# Autodesk Inventor assembly: v1.0
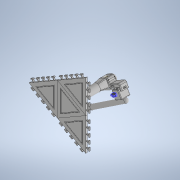
[picture p0: Inventor's stored thumbnail of the model, 180x180]
Saved by Autodesk Inventor 2022.3 (Build 263350000, 350)
## iProperties
Created: 2023-03-28
Part Number: v1.0
Document SubType Name: Assembly
Designer: Manuel Hueso Béjar
Author: Manuel Hueso Béjar
## Documents named in this file (13)
- C:\Users\Manuel Hueso Béjar\Desktop\3\2º Cuatrimestre\Robótica\Trabajo\v1.0\v1.0.iam
- C:\Users\Manuel Hueso Béjar\Desktop\3\2º Cuatrimestre\Robótica\Trabajo\v1.0\Base.ipt
- C:\Users\Manuel Hueso Béjar\Downloads\nema-17-motor-a-pasos-17hs4401-1-7amp-4kg-cm-1.snapshot.4\Nema 17 Motor a Pasos 17HS4401.iam
- C:\Users\Manuel Hueso Béjar\Desktop\3\2º Cuatrimestre\Robótica\Trabajo\v1.0\Base2.ipt
- C:\Users\Manuel Hueso Béjar\Desktop\3\2º Cuatrimestre\Robótica\Trabajo\v1.0\Tube_1.ipt
- C:\Users\Manuel Hueso Béjar\Desktop\3\2º Cuatrimestre\Robótica\Trabajo\v1.0\Tube_2.ipt
- C:\Users\Manuel Hueso Béjar\Desktop\3\2º Cuatrimestre\Robótica\Trabajo\v1.0\Joint_Tubes_1_2.ipt
- C:\Users\Manuel Hueso Béjar\Downloads\timing-pulley-gt2-16-teeth-5mm-bore-2.snapshot.7\GT2-16T\GT2_16T.ipt
- C:\Users\Manuel Hueso Béjar\Desktop\3\2º Cuatrimestre\Robótica\Trabajo\v1.0\Rod_1.ipt
- C:\Users\Manuel Hueso Béjar\Downloads\rolling-bearing-lmxxuu-1.snapshot.6\roulement lmxxuu (ap203).ipt
- C:\Users\Manuel Hueso Béjar\Desktop\3\2º Cuatrimestre\Robótica\Trabajo\v1.0\Joint_Bearings.ipt
- C:\Users\Manuel Hueso Béjar\Downloads\sg90-micro-servo-9g-tower-pro-1.snapshot.3\SG90 - Micro Servo 9g - Tower Pro.1.ipt
- C:\Users\Manuel Hueso Béjar\Desktop\3\2º Cuatrimestre\Robótica\Trabajo\v1.0\Tube_3.ipt
## Components (19 placed, 12 different names)
1. Base:1 — Rigid:1, Rigid:2, Rigid:3, Rigid:4, Rotational:7
2. Nema 17 Motor a Pasos 17HS4401:1 [sub-assembly] — Rigid:1
3. Base2:1 — Rigid:2
4. Base2:2 — Rigid:3
5. Base2:3 — Rigid:4
6. Tube_1:1 — Mate:3, Rigid:5, Mate:4, Mate:5, Mate:6, Mate:7, Rotational:7
7. Nema 17 Motor a Pasos 17HS4401:2 [sub-assembly] — Mate:8, Mate:9, Mate:10, Rotational:6
8. Nema 17 Motor a Pasos 17HS4401:3 [sub-assembly] — Mate:3, Rigid:5, Rotational:2
9. Tube_2:1 — Rotational:6, Rigid:8
10. Joint_Tubes_1_2:1 — Mate:4, Rotational:3, Rotational:4
11. GT2_16T:1 — Rotational:2
12. Joint_Tubes_1_2:2 — Mate:5, Mate:6, Mate:7, Rotational:5
13. Rod_1:1 — Rotational:4, Cylindrical:2
14. Rod_1:2 — Rotational:3, Rotational:5, Cylindrical:1
15. roulement lmxxuu (ap203):1 — Cylindrical:1, Rigid:7
16. roulement lmxxuu (ap203):2 — Cylindrical:2, Rigid:6
17. Joint_Bearings:1 — Rigid:6, Rigid:7, Mate:8, Mate:9, Mate:10
18. SG90 - Micro Servo 9g - Tower Pro.1:1
19. Tube_3:1 — Rigid:8
## Relationships (24: WeldJoint 8, Mate 8, RevoluteJoint 6, CylindricalJoint 2)
- Rigid:1 [WeldJoint]: Base:1 ↔ Nema 17 Motor a Pasos 17HS4401:1
- Rigid:2 [WeldJoint]: Base:1 ↔ Base2:1
- Rigid:3 [WeldJoint]: Base:1 ↔ Base2:2
- Rigid:4 [WeldJoint]: Base:1 ↔ Base2:3
- Mate:3: Tube_1:1 ↔ Nema 17 Motor a Pasos 17HS4401:3
- Rigid:5 [WeldJoint]: Tube_1:1 ↔ Nema 17 Motor a Pasos 17HS4401:3
- Rotational:2 [RevoluteJoint] (2.65 mm): Nema 17 Motor a Pasos 17HS4401:3 ↔ GT2_16T:1
- Mate:4: Tube_1:1 ↔ Joint_Tubes_1_2:1
- Mate:5: Tube_1:1 ↔ Joint_Tubes_1_2:2
- Mate:6: Tube_1:1 ↔ Joint_Tubes_1_2:2
- Mate:7: Tube_1:1 ↔ Joint_Tubes_1_2:2
- Rotational:3 [RevoluteJoint]: Joint_Tubes_1_2:1 ↔ Rod_1:2
- Rotational:4 [RevoluteJoint]: Joint_Tubes_1_2:1 ↔ Rod_1:1
- Rotational:5 [RevoluteJoint]: Joint_Tubes_1_2:2 ↔ Rod_1:2
- Cylindrical:1: Rod_1:2 ↔ roulement lmxxuu (ap203):1
- Cylindrical:2: Rod_1:1 ↔ roulement lmxxuu (ap203):2
- Rigid:6 [WeldJoint]: roulement lmxxuu (ap203):2 ↔ Joint_Bearings:1
- Rigid:7 [WeldJoint]: roulement lmxxuu (ap203):1 ↔ Joint_Bearings:1
- Mate:8: Nema 17 Motor a Pasos 17HS4401:2 ↔ Joint_Bearings:1
- Mate:9: Nema 17 Motor a Pasos 17HS4401:2 ↔ Joint_Bearings:1
- Mate:10: Nema 17 Motor a Pasos 17HS4401:2 ↔ Joint_Bearings:1
- Rotational:6 [RevoluteJoint]: Nema 17 Motor a Pasos 17HS4401:2 ↔ Tube_2:1
- Rigid:8 [WeldJoint]: Tube_2:1 ↔ Tube_3:1
- Rotational:7 [RevoluteJoint]: Base:1 ↔ Tube_1:1
